# Autodesk Inventor assembly: Vial Carousel
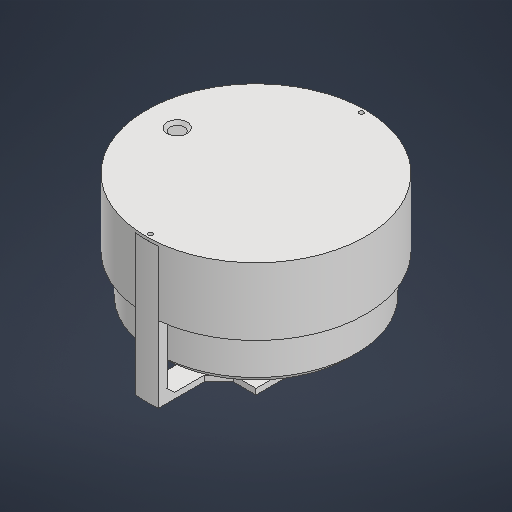
[picture p0: Inventor's stored thumbnail of the model, 512x512]
Saved by Autodesk Inventor 2025.1 (Build 291241000, 241)
## iProperties
Created: 2025-02-21
Part Number: Vial Carousel
Document SubType Name: Assembly
Designer: jerem
Author: jerem
## Documents named in this file (7)
- C:\Users\jerem\Documents\GitHub\Perovskite-Automated-Synthesis-System\CAD\vial carousel\Vial Carousel.iam
- C:\Users\jerem\Documents\GitHub\Perovskite-Automated-Synthesis-System\CAD\Non 3D Printed Parts\Motors and Servos\NEMA17 Stepper Motor - 26 mm.ipt
- C:\Users\jerem\Documents\GitHub\Perovskite-Automated-Synthesis-System\CAD\vial carousel\Vial Holder.ipt
- C:\Users\jerem\Documents\GitHub\Perovskite-Automated-Synthesis-System\CAD\Non 3D Printed Parts\Vial.ipt
- C:\Users\jerem\Documents\GitHub\Perovskite-Automated-Synthesis-System\CAD\vial carousel\Motor Mount.ipt
- C:\Users\jerem\Documents\GitHub\Perovskite-Automated-Synthesis-System\CAD\vial carousel\Shaft Collar.ipt
- C:\Users\jerem\Documents\GitHub\Perovskite-Automated-Synthesis-System\CAD\vial carousel\Vial Cover.ipt
## Components (8 placed, 6 different names)
1. NEMA17 Stepper Motor - 26 mm:1 — Mate:7, Mate:8, Mate:9, Mate:11, Mate:19, Mate:22
2. Vial Holder:1 — Mate:1, Mate:2, Mate:3, Mate:4, Mate:5, Mate:6, Mate:19, Mate:20, Mate:21
3. Vial:1 — Mate:4, Mate:5
4. Vial:2 — Mate:3, Mate:6
5. Vial:3 — Mate:1, Mate:2
6. Motor Mount:1 — Mate:7, Mate:8, Mate:9, Mate:15, Mate:16, Mate:17
7. Shaft Collar:1 — Mate:11, Mate:20, Mate:21, Mate:22
8. Vial Cover:1 — Mate:15, Mate:16, Mate:17
## Relationships (17: Mate 17)
- Mate:1: Vial Holder:1 ↔ Vial:3
- Mate:2: Vial Holder:1 ↔ Vial:3
- Mate:3: Vial Holder:1 ↔ Vial:2
- Mate:4: Vial Holder:1 ↔ Vial:1
- Mate:5: Vial Holder:1 ↔ Vial:1
- Mate:6: Vial Holder:1 ↔ Vial:2
- Mate:7: NEMA17 Stepper Motor - 26 mm:1 ↔ Motor Mount:1
- Mate:8: NEMA17 Stepper Motor - 26 mm:1 ↔ Motor Mount:1
- Mate:9: NEMA17 Stepper Motor - 26 mm:1 ↔ Motor Mount:1
- Mate:11: NEMA17 Stepper Motor - 26 mm:1 ↔ Shaft Collar:1
- Mate:15: Motor Mount:1 ↔ Vial Cover:1
- Mate:16: Motor Mount:1 ↔ Vial Cover:1
- Mate:17: Motor Mount:1 ↔ Vial Cover:1
- Mate:19: NEMA17 Stepper Motor - 26 mm:1 ↔ Vial Holder:1
- Mate:20: Vial Holder:1 ↔ Shaft Collar:1
- Mate:21: Vial Holder:1 ↔ Shaft Collar:1
- Mate:22: NEMA17 Stepper Motor - 26 mm:1 ↔ Shaft Collar:1
